# Autodesk Inventor assembly: Arm
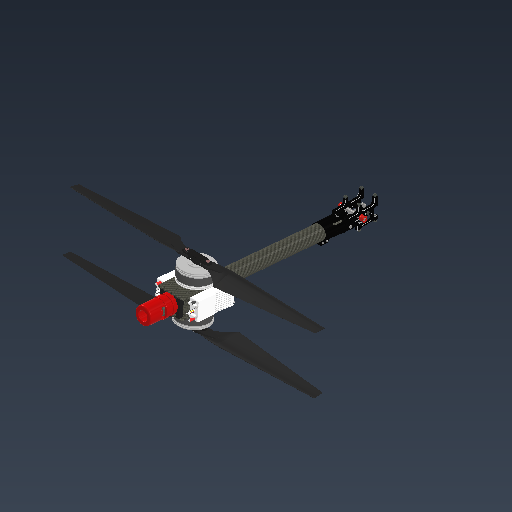
[picture p0: Inventor's stored thumbnail of the model, 512x512]
Saved by Autodesk Inventor 2024.1 (Build 281209000, 209)
## iProperties
Created: 2023-12-07
Part Number: Arm
Document SubType Name: Assembly
Designer: dzw04
Mass: 116.901 g
Surface Area: 623.445 cm^2
Volume: 52.4719 cm^3
Density: 2.22788 g/cm^3
Author: dzw04
## Documents named in this file (8)
- C:\Users\dzw04\Saxion\Mechatronica Lectoraat LMECH LED - Database ARG\Component_Database\SARAX\01. CAD\01. 3D_Drawing\02. Sub_Assemblies\Arm\Arm.iam
- C:\Users\dzw04\Saxion\Mechatronica Lectoraat LMECH LED - Database ARG\Component_Database\SARAX\01. CAD\01. 3D_Drawing\02. Sub_Assemblies\Z25_Folding_Arm\Z25_Folding_Arm.iam
- C:\Users\dzw04\Saxion\Mechatronica Lectoraat LMECH LED - Database ARG\Component_Database\SARAX\01. CAD\01. 3D_Drawing\02. Sub_Assemblies\Arm\01. Parts\Arm_Tube.ipt
- C:\Users\dzw04\Saxion\Mechatronica Lectoraat LMECH LED - Database ARG\Component_Database\SARAX\01. CAD\03. References\01. 3D_Files\Motor mount v12\Motor mount v12.iam
- C:\Users\dzw04\Saxion\Mechatronica Lectoraat LMECH LED - Database ARG\Component_Database\SARAX\01. CAD\03. References\01. 3D_Files\Arm bumper v3\Arm bumper v3.ipt
- C:\Users\dzw04\Saxion\Mechatronica Lectoraat LMECH LED - Database ARG\Component_Database\SARAX\01. CAD\03. References\01. 3D_Files\Motor mount v12\18x6-2F-CO-CCW v4 v3.iam
- C:\Users\dzw04\Saxion\Mechatronica Lectoraat LMECH LED - Database ARG\Component_Database\SARAX\01. CAD\01. 3D_Drawing\01. Parts\en-US\ISO 7380-1\ISO 7380-1 - M3 x 8.ipt
- C:\Users\dzw04\Saxion\Mechatronica Lectoraat LMECH LED - Database ARG\Component_Database\SARAX\01. CAD\01. 3D_Drawing\Parameters.xlsx
## Components (14 placed, 6 different names)
1. Z25_Folding_Arm:1 [sub-assembly] — Mate:1, Mate:2, Mate:3, Angle:1, Mate:11, Mate:12, Mate:13, Mate:14
2. Arm_Tube:1 — Mate:1, Mate:2, Mate:3, Mate:4, Flush:1, Mate:5, Mate:6
3. Motor mount v12:1 [sub-assembly] — Mate:4, Flush:1, Angle:1, Angle:2, Mate:7, Mate:8, Angle:3, Mate:9, Mate:10, Angle:4
4. Arm bumper v3:1 — Mate:5, Mate:6, Angle:2
5. 18x6-2F-CO-CCW v4 v3:1 [sub-assembly] — Mate:9, Mate:10, Angle:4
6. 18x6-2F-CO-CCW v4 v3:2 [sub-assembly] — Mate:7, Mate:8, Angle:3
7. ISO 7380-1 M3 x 8:2 — Mate:13, Mate:14
8. ISO 7380-1 M3 x 8:3
9. ISO 7380-1 M3 x 8:4
10. ISO 7380-1 M3 x 8:5
11. ISO 7380-1 M3 x 8:1 — Mate:11, Mate:12
12. ISO 7380-1 M3 x 8:6
13. ISO 7380-1 M3 x 8:7
14. ISO 7380-1 M3 x 8:8
## Component patterns: (4 elements, first: ISO 7380-1 M3 x 8:2), (4 elements, first: ISO 7380-1 M3 x 8:1)
## Relationships (19: Mate 14, Angle 4, Flush 1)
- Mate:1: Z25_Folding_Arm:1 ↔ Arm_Tube:1
- Mate:2: Z25_Folding_Arm:1 ↔ Arm_Tube:1
- Mate:3: Z25_Folding_Arm:1 ↔ Arm_Tube:1
- Mate:4: Arm_Tube:1 ↔ Motor mount v12:1
- Flush:1 (19 mm): Arm_Tube:1 ↔ Motor mount v12:1
- Angle:1 (0 deg): Z25_Folding_Arm:1 ↔ Motor mount v12:1
- Mate:5: Arm_Tube:1 ↔ Arm bumper v3:1
- Mate:6: Arm_Tube:1 ↔ Arm bumper v3:1
- Angle:2 (0 deg): Motor mount v12:1 ↔ Arm bumper v3:1
- Mate:7: Motor mount v12:1 ↔ 18x6-2F-CO-CCW v4 v3:2
- Mate:8: Motor mount v12:1 ↔ 18x6-2F-CO-CCW v4 v3:2
- Angle:3 (0 deg): Motor mount v12:1 ↔ 18x6-2F-CO-CCW v4 v3:2
- Mate:9: Motor mount v12:1 ↔ 18x6-2F-CO-CCW v4 v3:1
- Mate:10: Motor mount v12:1 ↔ 18x6-2F-CO-CCW v4 v3:1
- Angle:4 (0 deg): Motor mount v12:1 ↔ 18x6-2F-CO-CCW v4 v3:1
- Mate:11 (2 mm): Z25_Folding_Arm:1 ↔ ISO 7380-1 M3 x 8:1
- Mate:12: Z25_Folding_Arm:1 ↔ ISO 7380-1 M3 x 8:1
- Mate:13 (2 mm): Z25_Folding_Arm:1 ↔ ISO 7380-1 M3 x 8:2
- Mate:14: Z25_Folding_Arm:1 ↔ ISO 7380-1 M3 x 8:2
## Named parameters: BatteryLength = 200 mm, BatteryWidth = 62 mm, BatteryHeight = 76 mm, NumberofArms = 4, NumberOfArms = 4, RotorToRotor = 900 mm, MountToMotorCenter = 0 mm, LandingGearStabilityBar = 525 mm, LandingGearRod = 390 mm, ThicknessBatteryTopTray = 1 mm, ThicknessBatteryTray = 2 mm, ThicknessBodyCenterPlate = 2 mm, ThicknessLegLoadpipePlate = 2 mm, NumberOfBatterys = 2, ThicknessBodyOuterPlate = 2 mm, ArmPosition = 5 deg, LoadpipeLength = 450 mm, LandingGearHeight = 400 mm, StartAngleArm = 45 deg, MotorMountCenter = 71.5 mm
